# Autodesk Inventor assembly: Winch
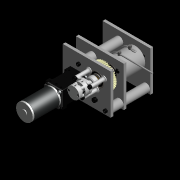
[picture p0: Inventor's stored thumbnail of the model, 180x180]
Saved by Autodesk Inventor 2014 SP1 (Build 180222100, 222)
## iProperties
Created: 2014-01-19
Part Number: Winch
Document SubType Name: Assembly
Designer: Rauhul Varma
Author: Rauhul Varma
## Documents named in this file (39)
- C:\Users\Rauhul Varma\Desktop\Winch Gearbox\Winch.iam
- C:\Users\Rauhul Varma\Desktop\Winch Gearbox\Plates\Motor Plate.ipt
- C:\Users\Rauhul Varma\Desktop\Winch Gearbox\Plates\Shifting Plate.ipt
- C:\Users\Rauhul Varma\Desktop\Winch Gearbox\Vex Versaplanetary 2 Stage Bag Motor.iam
- C:\Users\Rauhul Varma\Desktop\Winch Gearbox\Standoffs\Main Standoff.ipt
- C:\Users\Rauhul Varma\Desktop\Winch Gearbox\Ratchet.ipt
- C:\Users\Rauhul Varma\Desktop\Winch Gearbox\Bearings\R10-2RS.ipt
- C:\Users\Rauhul Varma\Desktop\Winch Gearbox\Bearings\FR8-2ZZ Hex.ipt
- C:\Users\Rauhul Varma\Desktop\Winch Gearbox\Gears\34T 20DP - .500 Hex Bore.ipt
- C:\Users\Rauhul Varma\Desktop\Winch Gearbox\Gears\44T 20DP - Ball Shifting Bore.ipt
- C:\Users\Rauhul Varma\Desktop\Winch Gearbox\Bearings\R10-Open.ipt
- C:\Users\Rauhul Varma\Desktop\Winch Gearbox\Bearings\Thrust Bearing Washer - .6250 Bore.ipt
- C:\Users\Rauhul Varma\Desktop\Winch Gearbox\Standoffs\Versa Spacer 1.ipt
- C:\Users\Rauhul Varma\Desktop\Winch Gearbox\Standoffs\Ratchet Spacer.ipt
- C:\Users\Rauhul Varma\Desktop\Winch Gearbox\Standoffs\Ratchet Spacer - Short.ipt
- C:\Users\Rauhul Varma\Desktop\Winch Gearbox\Bolts\Socket Head Cap Screw 10-32 Thread 1.500 Length.ipt
- C:\Users\Rauhul Varma\Desktop\Winch Gearbox\Bolts\Countersunk Socket Head Cap Screw 10-32 Thread .750 Length.ipt
- C:\Users\Rauhul Varma\Desktop\Winch Gearbox\Bolts\Button Head Cap Screw 10-32 Thread .250 Length.ipt
- C:\Users\Rauhul Varma\Desktop\Winch Gearbox\Pneumatic\Pancake Pneumatic.iam
- C:\Users\Rauhul Varma\Desktop\Winch Gearbox\Pneumatic\Pneumatic Hub.ipt
- C:\Users\Rauhul Varma\Desktop\Winch Gearbox\Bolts\Socket Head Cap Screw .25-20 Thread 1.500 Length.ipt
- C:\Users\Rauhul Varma\Desktop\Winch Gearbox\Standoffs\Pneumatic Standoff Curved.ipt
- C:\Users\Rauhul Varma\Desktop\Winch Gearbox\Plates\Pnuematic Plate.ipt
- C:\Users\Rauhul Varma\Desktop\Winch Gearbox\Bolts\Socket Head Cap Screw 4-40 Thread 1.125 Length.ipt
- C:\Users\Rauhul Varma\Desktop\Winch Gearbox\Pemnuts\4-40 Clinch Style Pem Nut .091 Minimum Panel Thickness.ipt
- C:\Users\Rauhul Varma\Desktop\Winch Gearbox\Plates\Winch Plate.ipt
- C:\Users\Rauhul Varma\Desktop\Winch Gearbox\Shafts\Winch Shaft.ipt
- C:\Users\Rauhul Varma\Desktop\Winch Gearbox\Shafts\Ball Shift.ipt
- C:\Users\Rauhul Varma\Desktop\Winch Gearbox\Shafts\Winch Shaft Bushing.ipt
- C:\Users\Rauhul Varma\Desktop\Winch Gearbox\Bolts\Button Head Cap Screw 4-40 Thread .125 Length.ipt
- C:\Users\Rauhul Varma\Desktop\Winch Gearbox\Bearings\R3-2RS.ipt
- C:\Users\Rauhul Varma\Desktop\Winch Gearbox\Shafts\Winch Body.ipt
- C:\Users\Rauhul Varma\Desktop\Winch Gearbox\Standoffs\Winch Standoff.ipt
- C:\Users\Rauhul Varma\Desktop\Winch Gearbox\Bolts\Socket Head Cap Screw 10-32 Thread 4.000 Length.ipt
- C:\Users\Rauhul Varma\Desktop\Winch Gearbox\Shafts\Winch Pin.ipt
- C:\Users\Rauhul Varma\Desktop\Winch Gearbox\Bolts\Socket Head Cap Screw 8-32 Thread .375 Length.ipt
- C:\Users\Rauhul Varma\Desktop\Winch Gearbox\Winch Coil.ipt
- C:\Users\Rauhul Varma\Desktop\Winch Gearbox\Winch Coil Revo.ipt
- C:\Users\Rauhul Varma\Desktop\Winch Gearbox\Winch Coil 2.ipt
## Components (62 placed, 38 different names)
1. Motor Plate:1 — Mate:1, Mate:2, Mate:3, Mate:5, Mate:6, Mate:8, Mate:9, Mate:10, Mate:11, Mate:13, Mate:18, Flush:2, Mate:33, Mate:34, Mate:43, Mate:46, Tangent:1, Tangent:2, Mate:57, Mate:58, Mate:60, Mate:61, Mate:62, Mate:63, Mate:64, Mate:65, Mate:119, Mate:120, Mate:121, Mate:122, Mate:123, Mate:124
2. Shifting Plate:1 — Mate:1, Mate:2, Mate:14, Mate:15, Mate:16, Mate:17, Mate:32, Mate:48, Mate:49, Mate:50, Mate:88, Mate:89, Flush:5, Mate:97, Mate:98, Mate:99, Mate:116, Mate:117, Mate:118, Angle:3, Angle:4
3. Vex Versaplanetary 2 Stage Bag Motor:1 [sub-assembly] — Mate:3, Mate:5, Angle:1, Mate:19, Angle:2, Mate:29, Mate:30, Mate:47
4. Main Standoff:1 — Mate:8, Mate:9, Mate:32, Mate:114
5. Main Standoff:2 — Mate:10, Mate:113
6. Main Standoff:3 — Mate:6, Mate:11, Mate:115
7. Ratchet:1 — Mate:13, Mate:14, Mate:31, Mate:35, Mate:36
8. R10-2RS:1 — Mate:17, Mate:21, Mate:22, Flush:5, Mate:103
9. R10-2RS:2 — Mate:18, Flush:2, Mate:24, Mate:25, Mate:28, Mate:54, Mate:100
10. FR8-2ZZ Hex:1 — Mate:15, Angle:1, Mate:16
11. 34T 20DP - .500 Hex Bore:1 — Mate:19, Angle:2, Flush:3, Mate:31
12. 44T 20DP - Ball Shifting Bore:1 — Mate:21, Flush:3, Mate:23, Mate:26
13. R10-Open:1 — Mate:22, Mate:23, Mate:27
14. Thrust Bearing Washer - .6250 Bore:1 — Mate:24, Mate:27
15. Thrust Bearing Washer - .6250 Bore:2 — Mate:25, Mate:26, Mate:28
16. Versa Spacer 1:1 — Mate:29, Mate:30
17. Ratchet Spacer:1 — Mate:33, Mate:34
18. Ratchet Spacer - Short:1 — Mate:35, Mate:36
19. Countersunk Socket Head Cap Screw 10-32 Thread .750 Length:1 — Mate:46, Tangent:1
20. Countersunk Socket Head Cap Screw 10-32 Thread .750 Length:2 — Mate:43, Tangent:2, Mate:47
21. Button Head Cap Screw 10-32 Thread .250 Length:1 — Mate:48, Mate:99
22. Button Head Cap Screw 10-32 Thread .250 Length:2 — Mate:49, Mate:98
23. Button Head Cap Screw 10-32 Thread .250 Length:3 — Mate:50, Mate:97
24. Pancake Pneumatic:1 [sub-assembly] — Mate:54, Mate:55, Mate:56, Mate:69, Mate:71, Mate:72, Mate:79, Mate:80, Mate:81, Mate:82, Mate:87
25. Pneumatic Hub:1 — Mate:55, Mate:56, Mate:100, Flush:8, Mate:130, Mate:131, Mate:132, Mate:133, Mate:134, Mate:135
26. Socket Head Cap Screw .25-20 Thread 1.500 Length:1 — Mate:57, Mate:58
27. Pneumatic Standoff Curved:1 — Mate:60, Mate:64, Mate:67
28. Pneumatic Standoff Curved:2 — Mate:61, Mate:63, Mate:68, Mate:70
29. Pneumatic Standoff Curved:3 — Mate:62, Mate:65, Mate:66
30. Pnuematic Plate:1 — Mate:66, Mate:67, Mate:68, Mate:69, Mate:70, Mate:71, Mate:72, Mate:73, Mate:74, Mate:75, Mate:76, Mate:77, Mate:78, Mate:83, Mate:84, Mate:87, Mate:101, Mate:102
31. Socket Head Cap Screw 10-32 Thread 1.500 Length:4 — Mate:75, Mate:78
32. Socket Head Cap Screw 10-32 Thread 1.500 Length:5 — Mate:74, Mate:76
33. Socket Head Cap Screw 10-32 Thread 1.500 Length:6 — Mate:73, Mate:77
34. Socket Head Cap Screw 4-40 Thread 1.125 Length:1 — Mate:80, Mate:82
35. Socket Head Cap Screw 4-40 Thread 1.125 Length:2 — Mate:79, Mate:81
36. 4-40 Clinch Style Pem Nut .091 Minimum Panel Thickness:1 — Mate:84, Mate:102
37. 4-40 Clinch Style Pem Nut .091 Minimum Panel Thickness:2 — Mate:83, Mate:101
38. Winch Plate:1 — Mate:88, Mate:89, Mate:90, Mate:91, Mate:92, Mate:93, Mate:94, Mate:95, Mate:96, Flush:4
39. Button Head Cap Screw 10-32 Thread .250 Length:4 — Mate:90, Mate:94
40. Button Head Cap Screw 10-32 Thread .250 Length:5 — Mate:91, Mate:93
41. Button Head Cap Screw 10-32 Thread .250 Length:6 — Mate:92, Mate:95
42. R10-2RS:3 — Mate:96, Flush:4, Mate:103, Mate:104, Flush:6, Mate:112
43. Winch Shaft:1 — Mate:104, Flush:6, Mate:106, Flush:7, Mate:111, Mate:125
44. Ball Shift:1 — Mate:105, Mate:107, Mate:108, Mate:109, Mate:110
45. Winch Shaft Bushing:1 — Mate:105, Mate:106, Flush:7
46. Button Head Cap Screw 4-40 Thread .125 Length:1 — Mate:109, Mate:110
47. R3-2RS:1 — Mate:107, Mate:108, Flush:8
48. Winch Standoff:1 — Mate:115, Mate:117
49. Winch Standoff:2 — Mate:114, Mate:118
50. Winch Standoff:3 — Mate:113, Mate:116
51. Socket Head Cap Screw 10-32 Thread 4.000 Length:1 — Mate:121, Mate:124
52. Socket Head Cap Screw 10-32 Thread 4.000 Length:2 — Mate:120, Mate:123
53. Socket Head Cap Screw 10-32 Thread 4.000 Length:3 — Mate:119, Mate:122
54. Winch Body:1 — Mate:111, Mate:112, Mate:125, Mate:126, Mate:127, Mate:128, Mate:129, Mate:138, Mate:139, Mate:141
55. Winch Pin:1 — Mate:127, Angle:3, Mate:128, Mate:140
56. Winch Pin:2 — Mate:126, Angle:4, Mate:129, Mate:136, Mate:137, Mate:142, Mate:143
57. Button Head Cap Screw 4-40 Thread .125 Length:2 — Mate:130, Mate:131
58. Button Head Cap Screw 4-40 Thread .125 Length:3 — Mate:132, Mate:133
59. Socket Head Cap Screw 8-32 Thread .375 Length:1 — Mate:134, Mate:135
60. Winch Coil:1 — Mate:136, Mate:137, Mate:138
61. Winch Coil Revo:1 — Mate:139, Mate:140
62. Winch Coil 2:1 — Mate:141, Mate:142, Mate:143
## Relationships (138: Mate 125, Flush 7, Angle 4, Tangent 2)
- Mate:1: Motor Plate:1 ↔ Shifting Plate:1
- Mate:2: Motor Plate:1 ↔ Shifting Plate:1
- Mate:3: Motor Plate:1 ↔ Vex Versaplanetary 2 Stage Bag Motor:1
- Mate:5: Motor Plate:1 ↔ Vex Versaplanetary 2 Stage Bag Motor:1
- Mate:6: Motor Plate:1 ↔ Main Standoff:3
- Mate:8: Motor Plate:1 ↔ Main Standoff:1
- Mate:9: Motor Plate:1 ↔ Main Standoff:1
- Mate:10: Motor Plate:1 ↔ Main Standoff:2
- Mate:11: Motor Plate:1 ↔ Main Standoff:3
- Mate:13: Motor Plate:1 ↔ Ratchet:1
- Mate:14: Shifting Plate:1 ↔ Ratchet:1
- Mate:15: Shifting Plate:1 ↔ FR8-2ZZ Hex:1
- Angle:1 (0 deg): Vex Versaplanetary 2 Stage Bag Motor:1 ↔ FR8-2ZZ Hex:1
- Mate:16: Shifting Plate:1 ↔ FR8-2ZZ Hex:1
- Mate:17: Shifting Plate:1 ↔ R10-2RS:1
- Mate:18: Motor Plate:1 ↔ R10-2RS:2
- Flush:2: Motor Plate:1 ↔ R10-2RS:2
- Mate:19: Vex Versaplanetary 2 Stage Bag Motor:1 ↔ 34T 20DP - .500 Hex Bore:1
- Angle:2 (0 deg): Vex Versaplanetary 2 Stage Bag Motor:1 ↔ 34T 20DP - .500 Hex Bore:1
- Mate:21: R10-2RS:1 ↔ 44T 20DP - Ball Shifting Bore:1
- Flush:3: 34T 20DP - .500 Hex Bore:1 ↔ 44T 20DP - Ball Shifting Bore:1
- Mate:22: R10-2RS:1 ↔ R10-Open:1
- Mate:23: 44T 20DP - Ball Shifting Bore:1 ↔ R10-Open:1
- Mate:24: R10-2RS:2 ↔ Thrust Bearing Washer - .6250 Bore:1
- Mate:25: R10-2RS:2 ↔ Thrust Bearing Washer - .6250 Bore:2
- Mate:26: 44T 20DP - Ball Shifting Bore:1 ↔ Thrust Bearing Washer - .6250 Bore:2
- Mate:27: R10-Open:1 ↔ Thrust Bearing Washer - .6250 Bore:1
- Mate:28: R10-2RS:2 ↔ Thrust Bearing Washer - .6250 Bore:2
- Mate:29: Vex Versaplanetary 2 Stage Bag Motor:1 ↔ Versa Spacer 1:1
- Mate:30: Vex Versaplanetary 2 Stage Bag Motor:1 ↔ Versa Spacer 1:1
- Mate:31: Ratchet:1 ↔ 34T 20DP - .500 Hex Bore:1
- Mate:32: Shifting Plate:1 ↔ Main Standoff:1
- Mate:33: Motor Plate:1 ↔ Ratchet Spacer:1
- Mate:34: Motor Plate:1 ↔ Ratchet Spacer:1
- Mate:35: Ratchet:1 ↔ Ratchet Spacer - Short:1
- Mate:36: Ratchet:1 ↔ Ratchet Spacer - Short:1
- Mate:43: Motor Plate:1 ↔ Countersunk Socket Head Cap Screw 10-32 Thread .750 Length:2
- Mate:46: Motor Plate:1 ↔ Countersunk Socket Head Cap Screw 10-32 Thread .750 Length:1
- Tangent:1: Motor Plate:1 ↔ Countersunk Socket Head Cap Screw 10-32 Thread .750 Length:1
- Tangent:2: Motor Plate:1 ↔ Countersunk Socket Head Cap Screw 10-32 Thread .750 Length:2
- Mate:47: Vex Versaplanetary 2 Stage Bag Motor:1 ↔ Countersunk Socket Head Cap Screw 10-32 Thread .750 Length:2
- Mate:48: Shifting Plate:1 ↔ Button Head Cap Screw 10-32 Thread .250 Length:1
- Mate:49: Shifting Plate:1 ↔ Button Head Cap Screw 10-32 Thread .250 Length:2
- Mate:50: Shifting Plate:1 ↔ Button Head Cap Screw 10-32 Thread .250 Length:3
- Mate:54: R10-2RS:2 ↔ Pancake Pneumatic:1
- Mate:55: Pancake Pneumatic:1 ↔ Pneumatic Hub:1
- Mate:56: Pancake Pneumatic:1 ↔ Pneumatic Hub:1
- Mate:57: Motor Plate:1 ↔ Socket Head Cap Screw .25-20 Thread 1.500 Length:1
- Mate:58: Motor Plate:1 ↔ Socket Head Cap Screw .25-20 Thread 1.500 Length:1
- Mate:60: Motor Plate:1 ↔ Pneumatic Standoff Curved:1
- Mate:61: Motor Plate:1 ↔ Pneumatic Standoff Curved:2
- Mate:62: Motor Plate:1 ↔ Pneumatic Standoff Curved:3
- Mate:63: Motor Plate:1 ↔ Pneumatic Standoff Curved:2
- Mate:64: Motor Plate:1 ↔ Pneumatic Standoff Curved:1
- Mate:65: Motor Plate:1 ↔ Pneumatic Standoff Curved:3
- Mate:66: Pneumatic Standoff Curved:3 ↔ Pnuematic Plate:1
- Mate:67: Pneumatic Standoff Curved:1 ↔ Pnuematic Plate:1
- Mate:68: Pneumatic Standoff Curved:2 ↔ Pnuematic Plate:1
- Mate:69: Pancake Pneumatic:1 ↔ Pnuematic Plate:1
- Mate:70: Pneumatic Standoff Curved:2 ↔ Pnuematic Plate:1
- Mate:71: Pancake Pneumatic:1 ↔ Pnuematic Plate:1
- Mate:72: Pancake Pneumatic:1 ↔ Pnuematic Plate:1
- Mate:73: Pnuematic Plate:1 ↔ Socket Head Cap Screw 10-32 Thread 1.500 Length:6
- Mate:74: Pnuematic Plate:1 ↔ Socket Head Cap Screw 10-32 Thread 1.500 Length:5
- Mate:75: Pnuematic Plate:1 ↔ Socket Head Cap Screw 10-32 Thread 1.500 Length:4
- Mate:76: Pnuematic Plate:1 ↔ Socket Head Cap Screw 10-32 Thread 1.500 Length:5
- Mate:77: Pnuematic Plate:1 ↔ Socket Head Cap Screw 10-32 Thread 1.500 Length:6
- Mate:78: Pnuematic Plate:1 ↔ Socket Head Cap Screw 10-32 Thread 1.500 Length:4
- Mate:79: Pancake Pneumatic:1 ↔ Socket Head Cap Screw 4-40 Thread 1.125 Length:2
- Mate:80: Pancake Pneumatic:1 ↔ Socket Head Cap Screw 4-40 Thread 1.125 Length:1
- Mate:81: Pancake Pneumatic:1 ↔ Socket Head Cap Screw 4-40 Thread 1.125 Length:2
- Mate:82: Pancake Pneumatic:1 ↔ Socket Head Cap Screw 4-40 Thread 1.125 Length:1
- Mate:83: Pnuematic Plate:1 ↔ 4-40 Clinch Style Pem Nut .091 Minimum Panel Thickness:2
- Mate:84: Pnuematic Plate:1 ↔ 4-40 Clinch Style Pem Nut .091 Minimum Panel Thickness:1
- Mate:87: Pancake Pneumatic:1 ↔ Pnuematic Plate:1
- Mate:88: Shifting Plate:1 ↔ Winch Plate:1
- Mate:89: Shifting Plate:1 ↔ Winch Plate:1
- Mate:90: Winch Plate:1 ↔ Button Head Cap Screw 10-32 Thread .250 Length:4
- Mate:91: Winch Plate:1 ↔ Button Head Cap Screw 10-32 Thread .250 Length:5
- Mate:92: Winch Plate:1 ↔ Button Head Cap Screw 10-32 Thread .250 Length:6
- Mate:93: Winch Plate:1 ↔ Button Head Cap Screw 10-32 Thread .250 Length:5
- Mate:94: Winch Plate:1 ↔ Button Head Cap Screw 10-32 Thread .250 Length:4
- Mate:95: Winch Plate:1 ↔ Button Head Cap Screw 10-32 Thread .250 Length:6
- Mate:96: Winch Plate:1 ↔ R10-2RS:3
- Flush:4: Winch Plate:1 ↔ R10-2RS:3
- Flush:5: Shifting Plate:1 ↔ R10-2RS:1
- Mate:97: Shifting Plate:1 ↔ Button Head Cap Screw 10-32 Thread .250 Length:3
- Mate:98: Shifting Plate:1 ↔ Button Head Cap Screw 10-32 Thread .250 Length:2
- Mate:99: Shifting Plate:1 ↔ Button Head Cap Screw 10-32 Thread .250 Length:1
- Mate:100 (5.4673 mm): R10-2RS:2 ↔ Pneumatic Hub:1
- Mate:101: Pnuematic Plate:1 ↔ 4-40 Clinch Style Pem Nut .091 Minimum Panel Thickness:2
- Mate:102: Pnuematic Plate:1 ↔ 4-40 Clinch Style Pem Nut .091 Minimum Panel Thickness:1
- Mate:103 (52.3875 mm): R10-2RS:1 ↔ R10-2RS:3
- Mate:104: R10-2RS:3 ↔ Winch Shaft:1
- Flush:6: R10-2RS:3 ↔ Winch Shaft:1
- Mate:105: Ball Shift:1 ↔ Winch Shaft Bushing:1
- Mate:106: Winch Shaft:1 ↔ Winch Shaft Bushing:1
- Flush:7: Winch Shaft:1 ↔ Winch Shaft Bushing:1
- Mate:107: Ball Shift:1 ↔ R3-2RS:1
- Mate:108: Ball Shift:1 ↔ R3-2RS:1
- Mate:109: Ball Shift:1 ↔ Button Head Cap Screw 4-40 Thread .125 Length:1
- Mate:110: Ball Shift:1 ↔ Button Head Cap Screw 4-40 Thread .125 Length:1
- Flush:8: Pneumatic Hub:1 ↔ R3-2RS:1
- Mate:111: Winch Shaft:1 ↔ Winch Body:1
- Mate:112: R10-2RS:3 ↔ Winch Body:1
- Mate:113: Main Standoff:2 ↔ Winch Standoff:3
- Mate:114: Main Standoff:1 ↔ Winch Standoff:2
- Mate:115: Main Standoff:3 ↔ Winch Standoff:1
- Mate:116: Shifting Plate:1 ↔ Winch Standoff:3
- Mate:117: Shifting Plate:1 ↔ Winch Standoff:1
- Mate:118: Shifting Plate:1 ↔ Winch Standoff:2
- Mate:119: Motor Plate:1 ↔ Socket Head Cap Screw 10-32 Thread 4.000 Length:3
- Mate:120: Motor Plate:1 ↔ Socket Head Cap Screw 10-32 Thread 4.000 Length:2
- Mate:121: Motor Plate:1 ↔ Socket Head Cap Screw 10-32 Thread 4.000 Length:1
- Mate:122: Motor Plate:1 ↔ Socket Head Cap Screw 10-32 Thread 4.000 Length:3
- Mate:123: Motor Plate:1 ↔ Socket Head Cap Screw 10-32 Thread 4.000 Length:2
- Mate:124: Motor Plate:1 ↔ Socket Head Cap Screw 10-32 Thread 4.000 Length:1
- Mate:125: Winch Shaft:1 ↔ Winch Body:1
- Mate:126: Winch Body:1 ↔ Winch Pin:2
- Mate:127: Winch Body:1 ↔ Winch Pin:1
- Angle:3 (0 deg): Shifting Plate:1 ↔ Winch Pin:1
- Angle:4 (0 deg): Shifting Plate:1 ↔ Winch Pin:2
- Mate:128: Winch Body:1 ↔ Winch Pin:1
- Mate:129: Winch Body:1 ↔ Winch Pin:2
- Mate:130: Pneumatic Hub:1 ↔ Button Head Cap Screw 4-40 Thread .125 Length:2
- Mate:131: Pneumatic Hub:1 ↔ Button Head Cap Screw 4-40 Thread .125 Length:2
- Mate:132: Pneumatic Hub:1 ↔ Button Head Cap Screw 4-40 Thread .125 Length:3
- Mate:133: Pneumatic Hub:1 ↔ Button Head Cap Screw 4-40 Thread .125 Length:3
- Mate:134: Pneumatic Hub:1 ↔ Socket Head Cap Screw 8-32 Thread .375 Length:1
- Mate:135: Pneumatic Hub:1 ↔ Socket Head Cap Screw 8-32 Thread .375 Length:1
- Mate:136: Winch Pin:2 ↔ Winch Coil:1
- Mate:137: Winch Pin:2 ↔ Winch Coil:1
- Mate:138: Winch Body:1 ↔ Winch Coil:1
- Mate:139: Winch Body:1 ↔ Winch Coil Revo:1
- Mate:140: Winch Pin:1 ↔ Winch Coil Revo:1
- Mate:141: Winch Body:1 ↔ Winch Coil 2:1
- Mate:142: Winch Pin:2 ↔ Winch Coil 2:1
- Mate:143: Winch Pin:2 ↔ Winch Coil 2:1
